# Autodesk Inventor assembly: COMPONENTS
(part 3 of 5)
- C:\Users\Zara\Documents\hera-cad\Node\SNAP V2 enclosure release - pack-n-go export\SNAP V2 enclosure release - pack-n-go export\Workspaces\Workspace\drawings\SNAP Ver2 pack-n-go\Workgroups\NotInProject\CAPAE830X1050D995DD305L335N_C237.ipt
- C:\Users\Zara\Documents\hera-cad\Node\SNAP V2 enclosure release - pack-n-go export\SNAP V2 enclosure release - pack-n-go export\Workspaces\Workspace\drawings\SNAP Ver2 pack-n-go\Workgroups\NotInProject\CAPAE830X1050D995DD305L335N_C244.ipt
- C:\Users\Zara\Documents\hera-cad\Node\SNAP V2 enclosure release - pack-n-go export\SNAP V2 enclosure release - pack-n-go export\Workspaces\Workspace\drawings\SNAP Ver2 pack-n-go\Workgroups\NotInProject\CAPAE830X1050D995DD305L335N_C253.ipt
- C:\Users\Zara\Documents\hera-cad\Node\SNAP V2 enclosure release - pack-n-go export\SNAP V2 enclosure release - pack-n-go export\Workspaces\Workspace\drawings\SNAP Ver2 pack-n-go\Workgroups\NotInProject\CAPAE830X1050D995DD305L335N_C262.ipt
- C:\Users\Zara\Documents\hera-cad\Node\SNAP V2 enclosure release - pack-n-go export\SNAP V2 enclosure release - pack-n-go export\Workspaces\Workspace\drawings\SNAP Ver2 pack-n-go\Workgroups\NotInProject\CAPMP7343X180N-ALT1_C402.ipt
- C:\Users\Zara\Documents\hera-cad\Node\SNAP V2 enclosure release - pack-n-go export\SNAP V2 enclosure release - pack-n-go export\Workspaces\Workspace\drawings\SNAP Ver2 pack-n-go\Workgroups\NotInProject\CAPMP7343X180N-ALT1_C413.ipt
- C:\Users\Zara\Documents\hera-cad\Node\SNAP V2 enclosure release - pack-n-go export\SNAP V2 enclosure release - pack-n-go export\Workspaces\Workspace\drawings\SNAP Ver2 pack-n-go\Workgroups\NotInProject\CAPMP7343X180N-ALT1_C400.ipt
- C:\Users\Zara\Documents\hera-cad\Node\SNAP V2 enclosure release - pack-n-go export\SNAP V2 enclosure release - pack-n-go export\Workspaces\Workspace\drawings\SNAP Ver2 pack-n-go\Workgroups\NotInProject\CAPMP7343X180N-ALT1_C401.ipt
- C:\Users\Zara\Documents\hera-cad\Node\SNAP V2 enclosure release - pack-n-go export\SNAP V2 enclosure release - pack-n-go export\Workspaces\Workspace\drawings\SNAP Ver2 pack-n-go\Workgroups\NotInProject\CAPMP7343X180N-ALT1_C206.ipt
- C:\Users\Zara\Documents\hera-cad\Node\SNAP V2 enclosure release - pack-n-go export\SNAP V2 enclosure release - pack-n-go export\Workspaces\Workspace\drawings\SNAP Ver2 pack-n-go\Workgroups\NotInProject\CAPMP7343X180N-ALT1_C207.ipt
- C:\Users\Zara\Documents\hera-cad\Node\SNAP V2 enclosure release - pack-n-go export\SNAP V2 enclosure release - pack-n-go export\Workspaces\Workspace\drawings\SNAP Ver2 pack-n-go\Workgroups\NotInProject\CAPC2012X140N_C419.ipt
- C:\Users\Zara\Documents\hera-cad\Node\SNAP V2 enclosure release - pack-n-go export\SNAP V2 enclosure release - pack-n-go export\Workspaces\Workspace\drawings\SNAP Ver2 pack-n-go\Workgroups\NotInProject\CAPC2012X140N_C420.ipt
- C:\Users\Zara\Documents\hera-cad\Node\SNAP V2 enclosure release - pack-n-go export\SNAP V2 enclosure release - pack-n-go export\Workspaces\Workspace\drawings\SNAP Ver2 pack-n-go\Workgroups\NotInProject\CAPC2012X140N_C410.ipt
- C:\Users\Zara\Documents\hera-cad\Node\SNAP V2 enclosure release - pack-n-go export\SNAP V2 enclosure release - pack-n-go export\Workspaces\Workspace\drawings\SNAP Ver2 pack-n-go\Workgroups\NotInProject\CAPC2012X140N_C418.ipt
- C:\Users\Zara\Documents\hera-cad\Node\SNAP V2 enclosure release - pack-n-go export\SNAP V2 enclosure release - pack-n-go export\Workspaces\Workspace\drawings\SNAP Ver2 pack-n-go\Workgroups\NotInProject\CAPC2012X140N_C417.ipt
- C:\Users\Zara\Documents\hera-cad\Node\SNAP V2 enclosure release - pack-n-go export\SNAP V2 enclosure release - pack-n-go export\Workspaces\Workspace\drawings\SNAP Ver2 pack-n-go\Workgroups\NotInProject\CAPC2012X140N_C416.ipt
- C:\Users\Zara\Documents\hera-cad\Node\SNAP V2 enclosure release - pack-n-go export\SNAP V2 enclosure release - pack-n-go export\Workspaces\Workspace\drawings\SNAP Ver2 pack-n-go\Workgroups\NotInProject\CAPC2012X140N_C415.ipt
- C:\Users\Zara\Documents\hera-cad\Node\SNAP V2 enclosure release - pack-n-go export\SNAP V2 enclosure release - pack-n-go export\Workspaces\Workspace\drawings\SNAP Ver2 pack-n-go\Workgroups\NotInProject\CAPC2012X140N_C412.ipt
- C:\Users\Zara\Documents\hera-cad\Node\SNAP V2 enclosure release - pack-n-go export\SNAP V2 enclosure release - pack-n-go export\Workspaces\Workspace\drawings\SNAP Ver2 pack-n-go\Workgroups\NotInProject\CAPC2012X140N_C411.ipt
- C:\Users\Zara\Documents\hera-cad\Node\SNAP V2 enclosure release - pack-n-go export\SNAP V2 enclosure release - pack-n-go export\Workspaces\Workspace\drawings\SNAP Ver2 pack-n-go\Workgroups\NotInProject\CAPC2012X140N_C408.ipt
- C:\Users\Zara\Documents\hera-cad\Node\SNAP V2 enclosure release - pack-n-go export\SNAP V2 enclosure release - pack-n-go export\Workspaces\Workspace\drawings\SNAP Ver2 pack-n-go\Workgroups\NotInProject\CAPC2012X140N_C409.ipt
- C:\Users\Zara\Documents\hera-cad\Node\SNAP V2 enclosure release - pack-n-go export\SNAP V2 enclosure release - pack-n-go export\Workspaces\Workspace\drawings\SNAP Ver2 pack-n-go\Workgroups\NotInProject\CAPC2012X140N_C404.ipt
- C:\Users\Zara\Documents\hera-cad\Node\SNAP V2 enclosure release - pack-n-go export\SNAP V2 enclosure release - pack-n-go export\Workspaces\Workspace\drawings\SNAP Ver2 pack-n-go\Workgroups\NotInProject\CAPC2012X140N_C407.ipt
- C:\Users\Zara\Documents\hera-cad\Node\SNAP V2 enclosure release - pack-n-go export\SNAP V2 enclosure release - pack-n-go export\Workspaces\Workspace\drawings\SNAP Ver2 pack-n-go\Workgroups\NotInProject\CAPC2012X140N_C406.ipt
- C:\Users\Zara\Documents\hera-cad\Node\SNAP V2 enclosure release - pack-n-go export\SNAP V2 enclosure release - pack-n-go export\Workspaces\Workspace\drawings\SNAP Ver2 pack-n-go\Workgroups\NotInProject\CAPC2012X140N_C405.ipt
- C:\Users\Zara\Documents\hera-cad\Node\SNAP V2 enclosure release - pack-n-go export\SNAP V2 enclosure release - pack-n-go export\Workspaces\Workspace\drawings\SNAP Ver2 pack-n-go\Workgroups\NotInProject\CAPC2012X140N_C403.ipt
- C:\Users\Zara\Documents\hera-cad\Node\SNAP V2 enclosure release - pack-n-go export\SNAP V2 enclosure release - pack-n-go export\Workspaces\Workspace\drawings\SNAP Ver2 pack-n-go\Workgroups\NotInProject\CAPC2012X140N_C209.ipt
- C:\Users\Zara\Documents\hera-cad\Node\SNAP V2 enclosure release - pack-n-go export\SNAP V2 enclosure release - pack-n-go export\Workspaces\Workspace\drawings\SNAP Ver2 pack-n-go\Workgroups\NotInProject\CAPC2012X140N_C210.ipt
- C:\Users\Zara\Documents\hera-cad\Node\SNAP V2 enclosure release - pack-n-go export\SNAP V2 enclosure release - pack-n-go export\Workspaces\Workspace\drawings\SNAP Ver2 pack-n-go\Workgroups\NotInProject\CAPC2012X140N_C211.ipt
- C:\Users\Zara\Documents\hera-cad\Node\SNAP V2 enclosure release - pack-n-go export\SNAP V2 enclosure release - pack-n-go export\Workspaces\Workspace\drawings\SNAP Ver2 pack-n-go\Workgroups\NotInProject\CAPC2012X140N_C272.ipt
- C:\Users\Zara\Documents\hera-cad\Node\SNAP V2 enclosure release - pack-n-go export\SNAP V2 enclosure release - pack-n-go export\Workspaces\Workspace\drawings\SNAP Ver2 pack-n-go\Workgroups\NotInProject\CAPC2012X140N_C274.ipt
- C:\Users\Zara\Documents\hera-cad\Node\SNAP V2 enclosure release - pack-n-go export\SNAP V2 enclosure release - pack-n-go export\Workspaces\Workspace\drawings\SNAP Ver2 pack-n-go\Workgroups\NotInProject\CAPC2012X140N_C294.ipt
- C:\Users\Zara\Documents\hera-cad\Node\SNAP V2 enclosure release - pack-n-go export\SNAP V2 enclosure release - pack-n-go export\Workspaces\Workspace\drawings\SNAP Ver2 pack-n-go\Workgroups\NotInProject\CAPC2012X140N_C296.ipt
- C:\Users\Zara\Documents\hera-cad\Node\SNAP V2 enclosure release - pack-n-go export\SNAP V2 enclosure release - pack-n-go export\Workspaces\Workspace\drawings\SNAP Ver2 pack-n-go\Workgroups\NotInProject\CAPC2012X140N_C133.ipt
- C:\Users\Zara\Documents\hera-cad\Node\SNAP V2 enclosure release - pack-n-go export\SNAP V2 enclosure release - pack-n-go export\Workspaces\Workspace\drawings\SNAP Ver2 pack-n-go\Workgroups\NotInProject\CAPC2012X140N_C130.ipt
- C:\Users\Zara\Documents\hera-cad\Node\SNAP V2 enclosure release - pack-n-go export\SNAP V2 enclosure release - pack-n-go export\Workspaces\Workspace\drawings\SNAP Ver2 pack-n-go\Workgroups\NotInProject\CAPC2012X140N_C126.ipt
- C:\Users\Zara\Documents\hera-cad\Node\SNAP V2 enclosure release - pack-n-go export\SNAP V2 enclosure release - pack-n-go export\Workspaces\Workspace\drawings\SNAP Ver2 pack-n-go\Workgroups\NotInProject\CAPC2012X140N_C125.ipt
- C:\Users\Zara\Documents\hera-cad\Node\SNAP V2 enclosure release - pack-n-go export\SNAP V2 enclosure release - pack-n-go export\Workspaces\Workspace\drawings\SNAP Ver2 pack-n-go\Workgroups\NotInProject\CAPC2012X140N_C122.ipt
- C:\Users\Zara\Documents\hera-cad\Node\SNAP V2 enclosure release - pack-n-go export\SNAP V2 enclosure release - pack-n-go export\Workspaces\Workspace\drawings\SNAP Ver2 pack-n-go\Workgroups\NotInProject\CAPC2012X140N_C118.ipt
- C:\Users\Zara\Documents\hera-cad\Node\SNAP V2 enclosure release - pack-n-go export\SNAP V2 enclosure release - pack-n-go export\Workspaces\Workspace\drawings\SNAP Ver2 pack-n-go\Workgroups\NotInProject\CAPC0603X30L_C278.ipt
- C:\Users\Zara\Documents\hera-cad\Node\SNAP V2 enclosure release - pack-n-go export\SNAP V2 enclosure release - pack-n-go export\Workspaces\Workspace\drawings\SNAP Ver2 pack-n-go\Workgroups\NotInProject\CAPC0603X30L_C281.ipt
- C:\Users\Zara\Documents\hera-cad\Node\SNAP V2 enclosure release - pack-n-go export\SNAP V2 enclosure release - pack-n-go export\Workspaces\Workspace\drawings\SNAP Ver2 pack-n-go\Workgroups\NotInProject\CAPC0603X30L_C283.ipt
- C:\Users\Zara\Documents\hera-cad\Node\SNAP V2 enclosure release - pack-n-go export\SNAP V2 enclosure release - pack-n-go export\Workspaces\Workspace\drawings\SNAP Ver2 pack-n-go\Workgroups\NotInProject\CAPC0603X30L_C288.ipt
- C:\Users\Zara\Documents\hera-cad\Node\SNAP V2 enclosure release - pack-n-go export\SNAP V2 enclosure release - pack-n-go export\Workspaces\Workspace\drawings\SNAP Ver2 pack-n-go\Workgroups\NotInProject\CAPC0603X30L_C300.ipt
- C:\Users\Zara\Documents\hera-cad\Node\SNAP V2 enclosure release - pack-n-go export\SNAP V2 enclosure release - pack-n-go export\Workspaces\Workspace\drawings\SNAP Ver2 pack-n-go\Workgroups\NotInProject\CAPC0603X30L_C303.ipt
- C:\Users\Zara\Documents\hera-cad\Node\SNAP V2 enclosure release - pack-n-go export\SNAP V2 enclosure release - pack-n-go export\Workspaces\Workspace\drawings\SNAP Ver2 pack-n-go\Workgroups\NotInProject\CAPC0603X30L_C305.ipt
- C:\Users\Zara\Documents\hera-cad\Node\SNAP V2 enclosure release - pack-n-go export\SNAP V2 enclosure release - pack-n-go export\Workspaces\Workspace\drawings\SNAP Ver2 pack-n-go\Workgroups\NotInProject\CAPC0603X30L_C310.ipt
- C:\Users\Zara\Documents\hera-cad\Node\SNAP V2 enclosure release - pack-n-go export\SNAP V2 enclosure release - pack-n-go export\Workspaces\Workspace\drawings\SNAP Ver2 pack-n-go\Workgroups\NotInProject\SOD3717X135_D10.ipt
- C:\Users\Zara\Documents\hera-cad\Node\SNAP V2 enclosure release - pack-n-go export\SNAP V2 enclosure release - pack-n-go export\Workspaces\Workspace\drawings\SNAP Ver2 pack-n-go\Workgroups\NotInProject\SOD3717X135_D9.ipt
- C:\Users\Zara\Documents\hera-cad\Node\SNAP V2 enclosure release - pack-n-go export\SNAP V2 enclosure release - pack-n-go export\Workspaces\Workspace\drawings\SNAP Ver2 pack-n-go\Workgroups\NotInProject\LEDM180X60X60N_DS1.ipt
- C:\Users\Zara\Documents\hera-cad\Node\SNAP V2 enclosure release - pack-n-go export\SNAP V2 enclosure release - pack-n-go export\Workspaces\Workspace\drawings\SNAP Ver2 pack-n-go\Workgroups\NotInProject\LEDM180X60X60N_DS10.ipt
- C:\Users\Zara\Documents\hera-cad\Node\SNAP V2 enclosure release - pack-n-go export\SNAP V2 enclosure release - pack-n-go export\Workspaces\Workspace\drawings\SNAP Ver2 pack-n-go\Workgroups\NotInProject\LEDM180X60X60N_DS11.ipt
- C:\Users\Zara\Documents\hera-cad\Node\SNAP V2 enclosure release - pack-n-go export\SNAP V2 enclosure release - pack-n-go export\Workspaces\Workspace\drawings\SNAP Ver2 pack-n-go\Workgroups\NotInProject\LEDM180X60X60N_DS4.ipt
- C:\Users\Zara\Documents\hera-cad\Node\SNAP V2 enclosure release - pack-n-go export\SNAP V2 enclosure release - pack-n-go export\Workspaces\Workspace\drawings\SNAP Ver2 pack-n-go\Workgroups\NotInProject\LEDM180X60X60N_DS5.ipt
- C:\Users\Zara\Documents\hera-cad\Node\SNAP V2 enclosure release - pack-n-go export\SNAP V2 enclosure release - pack-n-go export\Workspaces\Workspace\drawings\SNAP Ver2 pack-n-go\Workgroups\NotInProject\LEDM180X60X60N_DS7.ipt
- C:\Users\Zara\Documents\hera-cad\Node\SNAP V2 enclosure release - pack-n-go export\SNAP V2 enclosure release - pack-n-go export\Workspaces\Workspace\drawings\SNAP Ver2 pack-n-go\Workgroups\NotInProject\LEDM180X60X60N_DS8.ipt
- C:\Users\Zara\Documents\hera-cad\Node\SNAP V2 enclosure release - pack-n-go export\SNAP V2 enclosure release - pack-n-go export\Workspaces\Workspace\drawings\SNAP Ver2 pack-n-go\Workgroups\NotInProject\LEDM180X60X60N_DS9.ipt
- C:\Users\Zara\Documents\hera-cad\Node\SNAP V2 enclosure release - pack-n-go export\SNAP V2 enclosure release - pack-n-go export\Workspaces\Workspace\drawings\SNAP Ver2 pack-n-go\Workgroups\NotInProject\LEDM180X60X60N_DS2.ipt
- C:\Users\Zara\Documents\hera-cad\Node\SNAP V2 enclosure release - pack-n-go export\SNAP V2 enclosure release - pack-n-go export\Workspaces\Workspace\drawings\SNAP Ver2 pack-n-go\Workgroups\NotInProject\LEDM180X60X60N_DS3.ipt
- C:\Users\Zara\Documents\hera-cad\Node\SNAP V2 enclosure release - pack-n-go export\SNAP V2 enclosure release - pack-n-go export\Workspaces\Workspace\drawings\SNAP Ver2 pack-n-go\Workgroups\NotInProject\INDM4532X340N_L1.ipt
- C:\Users\Zara\Documents\hera-cad\Node\SNAP V2 enclosure release - pack-n-go export\SNAP V2 enclosure release - pack-n-go export\Workspaces\Workspace\drawings\SNAP Ver2 pack-n-go\Workgroups\NotInProject\INDM4532X340N_L10.ipt
- C:\Users\Zara\Documents\hera-cad\Node\SNAP V2 enclosure release - pack-n-go export\SNAP V2 enclosure release - pack-n-go export\Workspaces\Workspace\drawings\SNAP Ver2 pack-n-go\Workgroups\NotInProject\INDM4532X340N_L11.ipt
- C:\Users\Zara\Documents\hera-cad\Node\SNAP V2 enclosure release - pack-n-go export\SNAP V2 enclosure release - pack-n-go export\Workspaces\Workspace\drawings\SNAP Ver2 pack-n-go\Workgroups\NotInProject\INDM4532X340N_L12.ipt
- C:\Users\Zara\Documents\hera-cad\Node\SNAP V2 enclosure release - pack-n-go export\SNAP V2 enclosure release - pack-n-go export\Workspaces\Workspace\drawings\SNAP Ver2 pack-n-go\Workgroups\NotInProject\INDM4532X340N_L2.ipt
- C:\Users\Zara\Documents\hera-cad\Node\SNAP V2 enclosure release - pack-n-go export\SNAP V2 enclosure release - pack-n-go export\Workspaces\Workspace\drawings\SNAP Ver2 pack-n-go\Workgroups\NotInProject\INDM4532X340N_L3.ipt
- C:\Users\Zara\Documents\hera-cad\Node\SNAP V2 enclosure release - pack-n-go export\SNAP V2 enclosure release - pack-n-go export\Workspaces\Workspace\drawings\SNAP Ver2 pack-n-go\Workgroups\NotInProject\INDM4532X340N_L4.ipt
- C:\Users\Zara\Documents\hera-cad\Node\SNAP V2 enclosure release - pack-n-go export\SNAP V2 enclosure release - pack-n-go export\Workspaces\Workspace\drawings\SNAP Ver2 pack-n-go\Workgroups\NotInProject\INDM4532X340N_L5.ipt
- C:\Users\Zara\Documents\hera-cad\Node\SNAP V2 enclosure release - pack-n-go export\SNAP V2 enclosure release - pack-n-go export\Workspaces\Workspace\drawings\SNAP Ver2 pack-n-go\Workgroups\NotInProject\INDM4532X340N_L6.ipt
- C:\Users\Zara\Documents\hera-cad\Node\SNAP V2 enclosure release - pack-n-go export\SNAP V2 enclosure release - pack-n-go export\Workspaces\Workspace\drawings\SNAP Ver2 pack-n-go\Workgroups\NotInProject\INDM4532X340N_L8.ipt
- C:\Users\Zara\Documents\hera-cad\Node\SNAP V2 enclosure release - pack-n-go export\SNAP V2 enclosure release - pack-n-go export\Workspaces\Workspace\drawings\SNAP Ver2 pack-n-go\Workgroups\NotInProject\INDM4532X340N_L7.ipt
- C:\Users\Zara\Documents\hera-cad\Node\SNAP V2 enclosure release - pack-n-go export\SNAP V2 enclosure release - pack-n-go export\Workspaces\Workspace\drawings\SNAP Ver2 pack-n-go\Workgroups\NotInProject\INDM4532X340N_L9.ipt
- C:\Users\Zara\Documents\hera-cad\Node\SNAP V2 enclosure release - pack-n-go export\SNAP V2 enclosure release - pack-n-go export\Workspaces\Workspace\drawings\SNAP Ver2 pack-n-go\Workgroups\NotInProject\INDC2012X110N_L14.ipt
- C:\Users\Zara\Documents\hera-cad\Node\SNAP V2 enclosure release - pack-n-go export\SNAP V2 enclosure release - pack-n-go export\Workspaces\Workspace\drawings\SNAP Ver2 pack-n-go\Workgroups\NotInProject\INDC2012X110N_L13.ipt
- C:\Users\Zara\Documents\hera-cad\Node\SNAP V2 enclosure release - pack-n-go export\SNAP V2 enclosure release - pack-n-go export\Workspaces\Workspace\drawings\SNAP Ver2 pack-n-go\Workgroups\NotInProject\INDM9630X305N_L15.ipt
- C:\Users\Zara\Documents\hera-cad\Node\SNAP V2 enclosure release - pack-n-go export\SNAP V2 enclosure release - pack-n-go export\Workspaces\Workspace\drawings\SNAP Ver2 pack-n-go\Workgroups\NotInProject\INDM9630X305N_L16.ipt
- C:\Users\Zara\Documents\hera-cad\Node\SNAP V2 enclosure release - pack-n-go export\SNAP V2 enclosure release - pack-n-go export\Workspaces\Workspace\drawings\SNAP Ver2 pack-n-go\Workgroups\NotInProject\INDM9630X305N_L17.ipt
- C:\Users\Zara\Documents\hera-cad\Node\SNAP V2 enclosure release - pack-n-go export\SNAP V2 enclosure release - pack-n-go export\Workspaces\Workspace\drawings\SNAP Ver2 pack-n-go\Workgroups\NotInProject\INDM9630X305N_L18.ipt
- C:\Users\Zara\Documents\hera-cad\Node\SNAP V2 enclosure release - pack-n-go export\SNAP V2 enclosure release - pack-n-go export\Workspaces\Workspace\drawings\SNAP Ver2 pack-n-go\Workgroups\NotInProject\INDM9630X305N_L19.ipt
- C:\Users\Zara\Documents\hera-cad\Node\SNAP V2 enclosure release - pack-n-go export\SNAP V2 enclosure release - pack-n-go export\Workspaces\Workspace\drawings\SNAP Ver2 pack-n-go\Workgroups\NotInProject\INDC1608X95L-ALT1_L20.ipt
- C:\Users\Zara\Documents\hera-cad\Node\SNAP V2 enclosure release - pack-n-go export\SNAP V2 enclosure release - pack-n-go export\Workspaces\Workspace\drawings\SNAP Ver2 pack-n-go\Workgroups\NotInProject\INDC1608X95L-ALT1_L21.ipt
- C:\Users\Zara\Documents\hera-cad\Node\SNAP V2 enclosure release - pack-n-go export\SNAP V2 enclosure release - pack-n-go export\Workspaces\Workspace\drawings\SNAP Ver2 pack-n-go\Workgroups\NotInProject\INDC1608X95L-ALT1_L23.ipt
- C:\Users\Zara\Documents\hera-cad\Node\SNAP V2 enclosure release - pack-n-go export\SNAP V2 enclosure release - pack-n-go export\Workspaces\Workspace\drawings\SNAP Ver2 pack-n-go\Workgroups\NotInProject\INDC1608X95L-ALT1_L22.ipt
- C:\Users\Zara\Documents\hera-cad\Node\SNAP V2 enclosure release - pack-n-go export\SNAP V2 enclosure release - pack-n-go export\Workspaces\Workspace\drawings\SNAP Ver2 pack-n-go\Workgroups\NotInProject\INDM5551X200N_L24.ipt
- C:\Users\Zara\Documents\hera-cad\Node\SNAP V2 enclosure release - pack-n-go export\SNAP V2 enclosure release - pack-n-go export\Workspaces\Workspace\drawings\SNAP Ver2 pack-n-go\Workgroups\NotInProject\INDM5551X200N_L25.ipt
- C:\Users\Zara\Documents\hera-cad\Node\SNAP V2 enclosure release - pack-n-go export\SNAP V2 enclosure release - pack-n-go export\Workspaces\Workspace\drawings\SNAP Ver2 pack-n-go\Workgroups\NotInProject\INDM5551X200N_L26.ipt
- C:\Users\Zara\Documents\hera-cad\Node\SNAP V2 enclosure release - pack-n-go export\SNAP V2 enclosure release - pack-n-go export\Workspaces\Workspace\drawings\SNAP Ver2 pack-n-go\Workgroups\NotInProject\INDM5551X200N_L27.ipt
- C:\Users\Zara\Documents\hera-cad\Node\SNAP V2 enclosure release - pack-n-go export\SNAP V2 enclosure release - pack-n-go export\Workspaces\Workspace\drawings\SNAP Ver2 pack-n-go\Workgroups\NotInProject\RESC1005X35N_R443.ipt
- C:\Users\Zara\Documents\hera-cad\Node\SNAP V2 enclosure release - pack-n-go export\SNAP V2 enclosure release - pack-n-go export\Workspaces\Workspace\drawings\SNAP Ver2 pack-n-go\Workgroups\NotInProject\RESC1005X35N_R442.ipt
- C:\Users\Zara\Documents\hera-cad\Node\SNAP V2 enclosure release - pack-n-go export\SNAP V2 enclosure release - pack-n-go export\Workspaces\Workspace\drawings\SNAP Ver2 pack-n-go\Workgroups\NotInProject\RESC1005X35N_R438.ipt
- C:\Users\Zara\Documents\hera-cad\Node\SNAP V2 enclosure release - pack-n-go export\SNAP V2 enclosure release - pack-n-go export\Workspaces\Workspace\drawings\SNAP Ver2 pack-n-go\Workgroups\NotInProject\RESC1005X35N_R437.ipt
- C:\Users\Zara\Documents\hera-cad\Node\SNAP V2 enclosure release - pack-n-go export\SNAP V2 enclosure release - pack-n-go export\Workspaces\Workspace\drawings\SNAP Ver2 pack-n-go\Workgroups\NotInProject\RESC1005X35N_R436.ipt
- C:\Users\Zara\Documents\hera-cad\Node\SNAP V2 enclosure release - pack-n-go export\SNAP V2 enclosure release - pack-n-go export\Workspaces\Workspace\drawings\SNAP Ver2 pack-n-go\Workgroups\NotInProject\RESC1005X35N_R434.ipt
- C:\Users\Zara\Documents\hera-cad\Node\SNAP V2 enclosure release - pack-n-go export\SNAP V2 enclosure release - pack-n-go export\Workspaces\Workspace\drawings\SNAP Ver2 pack-n-go\Workgroups\NotInProject\RESC1005X35N_R114.ipt
- C:\Users\Zara\Documents\hera-cad\Node\SNAP V2 enclosure release - pack-n-go export\SNAP V2 enclosure release - pack-n-go export\Workspaces\Workspace\drawings\SNAP Ver2 pack-n-go\Workgroups\NotInProject\RESC1005X35N_R133.ipt
- C:\Users\Zara\Documents\hera-cad\Node\SNAP V2 enclosure release - pack-n-go export\SNAP V2 enclosure release - pack-n-go export\Workspaces\Workspace\drawings\SNAP Ver2 pack-n-go\Workgroups\NotInProject\RESC1005X35N_R135.ipt
- C:\Users\Zara\Documents\hera-cad\Node\SNAP V2 enclosure release - pack-n-go export\SNAP V2 enclosure release - pack-n-go export\Workspaces\Workspace\drawings\SNAP Ver2 pack-n-go\Workgroups\NotInProject\RESC1005X35N_R139.ipt
- C:\Users\Zara\Documents\hera-cad\Node\SNAP V2 enclosure release - pack-n-go export\SNAP V2 enclosure release - pack-n-go export\Workspaces\Workspace\drawings\SNAP Ver2 pack-n-go\Workgroups\NotInProject\RESC1005X35N_R432.ipt
- C:\Users\Zara\Documents\hera-cad\Node\SNAP V2 enclosure release - pack-n-go export\SNAP V2 enclosure release - pack-n-go export\Workspaces\Workspace\drawings\SNAP Ver2 pack-n-go\Workgroups\NotInProject\RESC1005X35N_R431.ipt
- C:\Users\Zara\Documents\hera-cad\Node\SNAP V2 enclosure release - pack-n-go export\SNAP V2 enclosure release - pack-n-go export\Workspaces\Workspace\drawings\SNAP Ver2 pack-n-go\Workgroups\NotInProject\RESC1005X35N_R427.ipt
- C:\Users\Zara\Documents\hera-cad\Node\SNAP V2 enclosure release - pack-n-go export\SNAP V2 enclosure release - pack-n-go export\Workspaces\Workspace\drawings\SNAP Ver2 pack-n-go\Workgroups\NotInProject\RESC1005X35N_R426.ipt
- C:\Users\Zara\Documents\hera-cad\Node\SNAP V2 enclosure release - pack-n-go export\SNAP V2 enclosure release - pack-n-go export\Workspaces\Workspace\drawings\SNAP Ver2 pack-n-go\Workgroups\NotInProject\RESC1005X35N_R424.ipt
- C:\Users\Zara\Documents\hera-cad\Node\SNAP V2 enclosure release - pack-n-go export\SNAP V2 enclosure release - pack-n-go export\Workspaces\Workspace\drawings\SNAP Ver2 pack-n-go\Workgroups\NotInProject\RESC1005X35N_R423.ipt
- C:\Users\Zara\Documents\hera-cad\Node\SNAP V2 enclosure release - pack-n-go export\SNAP V2 enclosure release - pack-n-go export\Workspaces\Workspace\drawings\SNAP Ver2 pack-n-go\Workgroups\NotInProject\RESC1005X35N_R421.ipt
- C:\Users\Zara\Documents\hera-cad\Node\SNAP V2 enclosure release - pack-n-go export\SNAP V2 enclosure release - pack-n-go export\Workspaces\Workspace\drawings\SNAP Ver2 pack-n-go\Workgroups\NotInProject\RESC1005X35N_R420.ipt
- C:\Users\Zara\Documents\hera-cad\Node\SNAP V2 enclosure release - pack-n-go export\SNAP V2 enclosure release - pack-n-go export\Workspaces\Workspace\drawings\SNAP Ver2 pack-n-go\Workgroups\NotInProject\RESC1005X35N_R433.ipt
- C:\Users\Zara\Documents\hera-cad\Node\SNAP V2 enclosure release - pack-n-go export\SNAP V2 enclosure release - pack-n-go export\Workspaces\Workspace\drawings\SNAP Ver2 pack-n-go\Workgroups\NotInProject\RESC1005X35N_R428.ipt
- C:\Users\Zara\Documents\hera-cad\Node\SNAP V2 enclosure release - pack-n-go export\SNAP V2 enclosure release - pack-n-go export\Workspaces\Workspace\drawings\SNAP Ver2 pack-n-go\Workgroups\NotInProject\RESC1005X35N_R425.ipt
- C:\Users\Zara\Documents\hera-cad\Node\SNAP V2 enclosure release - pack-n-go export\SNAP V2 enclosure release - pack-n-go export\Workspaces\Workspace\drawings\SNAP Ver2 pack-n-go\Workgroups\NotInProject\RESC1005X35N_R422.ipt
- C:\Users\Zara\Documents\hera-cad\Node\SNAP V2 enclosure release - pack-n-go export\SNAP V2 enclosure release - pack-n-go export\Workspaces\Workspace\drawings\SNAP Ver2 pack-n-go\Workgroups\NotInProject\RESC1005X35N_R1.ipt
- C:\Users\Zara\Documents\hera-cad\Node\SNAP V2 enclosure release - pack-n-go export\SNAP V2 enclosure release - pack-n-go export\Workspaces\Workspace\drawings\SNAP Ver2 pack-n-go\Workgroups\NotInProject\RESC1005X35N_R12.ipt
- C:\Users\Zara\Documents\hera-cad\Node\SNAP V2 enclosure release - pack-n-go export\SNAP V2 enclosure release - pack-n-go export\Workspaces\Workspace\drawings\SNAP Ver2 pack-n-go\Workgroups\NotInProject\RESC1005X35N_R13.ipt
- C:\Users\Zara\Documents\hera-cad\Node\SNAP V2 enclosure release - pack-n-go export\SNAP V2 enclosure release - pack-n-go export\Workspaces\Workspace\drawings\SNAP Ver2 pack-n-go\Workgroups\NotInProject\RESC1005X35N_R16.ipt
- C:\Users\Zara\Documents\hera-cad\Node\SNAP V2 enclosure release - pack-n-go export\SNAP V2 enclosure release - pack-n-go export\Workspaces\Workspace\drawings\SNAP Ver2 pack-n-go\Workgroups\NotInProject\RESC1005X35N_R21.ipt
- C:\Users\Zara\Documents\hera-cad\Node\SNAP V2 enclosure release - pack-n-go export\SNAP V2 enclosure release - pack-n-go export\Workspaces\Workspace\drawings\SNAP Ver2 pack-n-go\Workgroups\NotInProject\RESC1005X35N_R25.ipt
- C:\Users\Zara\Documents\hera-cad\Node\SNAP V2 enclosure release - pack-n-go export\SNAP V2 enclosure release - pack-n-go export\Workspaces\Workspace\drawings\SNAP Ver2 pack-n-go\Workgroups\NotInProject\RESC1005X35N_R26.ipt
- C:\Users\Zara\Documents\hera-cad\Node\SNAP V2 enclosure release - pack-n-go export\SNAP V2 enclosure release - pack-n-go export\Workspaces\Workspace\drawings\SNAP Ver2 pack-n-go\Workgroups\NotInProject\RESC1005X35N_R28.ipt
- C:\Users\Zara\Documents\hera-cad\Node\SNAP V2 enclosure release - pack-n-go export\SNAP V2 enclosure release - pack-n-go export\Workspaces\Workspace\drawings\SNAP Ver2 pack-n-go\Workgroups\NotInProject\RESC1005X35N_R29.ipt
- C:\Users\Zara\Documents\hera-cad\Node\SNAP V2 enclosure release - pack-n-go export\SNAP V2 enclosure release - pack-n-go export\Workspaces\Workspace\drawings\SNAP Ver2 pack-n-go\Workgroups\NotInProject\RESC1005X35N_R32.ipt
- C:\Users\Zara\Documents\hera-cad\Node\SNAP V2 enclosure release - pack-n-go export\SNAP V2 enclosure release - pack-n-go export\Workspaces\Workspace\drawings\SNAP Ver2 pack-n-go\Workgroups\NotInProject\RESC1005X35N_R33.ipt
- C:\Users\Zara\Documents\hera-cad\Node\SNAP V2 enclosure release - pack-n-go export\SNAP V2 enclosure release - pack-n-go export\Workspaces\Workspace\drawings\SNAP Ver2 pack-n-go\Workgroups\NotInProject\RESC1005X35N_R36.ipt
- C:\Users\Zara\Documents\hera-cad\Node\SNAP V2 enclosure release - pack-n-go export\SNAP V2 enclosure release - pack-n-go export\Workspaces\Workspace\drawings\SNAP Ver2 pack-n-go\Workgroups\NotInProject\RESC1005X35N_R41.ipt
- C:\Users\Zara\Documents\hera-cad\Node\SNAP V2 enclosure release - pack-n-go export\SNAP V2 enclosure release - pack-n-go export\Workspaces\Workspace\drawings\SNAP Ver2 pack-n-go\Workgroups\NotInProject\RESC1005X35N_R45.ipt
- C:\Users\Zara\Documents\hera-cad\Node\SNAP V2 enclosure release - pack-n-go export\SNAP V2 enclosure release - pack-n-go export\Workspaces\Workspace\drawings\SNAP Ver2 pack-n-go\Workgroups\NotInProject\RESC1005X35N_R46.ipt
- C:\Users\Zara\Documents\hera-cad\Node\SNAP V2 enclosure release - pack-n-go export\SNAP V2 enclosure release - pack-n-go export\Workspaces\Workspace\drawings\SNAP Ver2 pack-n-go\Workgroups\NotInProject\RESC1005X35N_R48.ipt
- C:\Users\Zara\Documents\hera-cad\Node\SNAP V2 enclosure release - pack-n-go export\SNAP V2 enclosure release - pack-n-go export\Workspaces\Workspace\drawings\SNAP Ver2 pack-n-go\Workgroups\NotInProject\RESC1005X35N_R49.ipt
- C:\Users\Zara\Documents\hera-cad\Node\SNAP V2 enclosure release - pack-n-go export\SNAP V2 enclosure release - pack-n-go export\Workspaces\Workspace\drawings\SNAP Ver2 pack-n-go\Workgroups\NotInProject\RESC1005X35N_R5.ipt
- C:\Users\Zara\Documents\hera-cad\Node\SNAP V2 enclosure release - pack-n-go export\SNAP V2 enclosure release - pack-n-go export\Workspaces\Workspace\drawings\SNAP Ver2 pack-n-go\Workgroups\NotInProject\RESC1005X35N_R52.ipt
- C:\Users\Zara\Documents\hera-cad\Node\SNAP V2 enclosure release - pack-n-go export\SNAP V2 enclosure release - pack-n-go export\Workspaces\Workspace\drawings\SNAP Ver2 pack-n-go\Workgroups\NotInProject\RESC1005X35N_R53.ipt
- C:\Users\Zara\Documents\hera-cad\Node\SNAP V2 enclosure release - pack-n-go export\SNAP V2 enclosure release - pack-n-go export\Workspaces\Workspace\drawings\SNAP Ver2 pack-n-go\Workgroups\NotInProject\RESC1005X35N_R56.ipt
- C:\Users\Zara\Documents\hera-cad\Node\SNAP V2 enclosure release - pack-n-go export\SNAP V2 enclosure release - pack-n-go export\Workspaces\Workspace\drawings\SNAP Ver2 pack-n-go\Workgroups\NotInProject\RESC1005X35N_R6.ipt
- C:\Users\Zara\Documents\hera-cad\Node\SNAP V2 enclosure release - pack-n-go export\SNAP V2 enclosure release - pack-n-go export\Workspaces\Workspace\drawings\SNAP Ver2 pack-n-go\Workgroups\NotInProject\RESC1005X35N_R8.ipt
- C:\Users\Zara\Documents\hera-cad\Node\SNAP V2 enclosure release - pack-n-go export\SNAP V2 enclosure release - pack-n-go export\Workspaces\Workspace\drawings\SNAP Ver2 pack-n-go\Workgroups\NotInProject\RESC1005X35N_R9.ipt
- C:\Users\Zara\Documents\hera-cad\Node\SNAP V2 enclosure release - pack-n-go export\SNAP V2 enclosure release - pack-n-go export\Workspaces\Workspace\drawings\SNAP Ver2 pack-n-go\Workgroups\NotInProject\RESC1005X35N_R10.ipt
- C:\Users\Zara\Documents\hera-cad\Node\SNAP V2 enclosure release - pack-n-go export\SNAP V2 enclosure release - pack-n-go export\Workspaces\Workspace\drawings\SNAP Ver2 pack-n-go\Workgroups\NotInProject\RESC1005X35N_R14.ipt
- C:\Users\Zara\Documents\hera-cad\Node\SNAP V2 enclosure release - pack-n-go export\SNAP V2 enclosure release - pack-n-go export\Workspaces\Workspace\drawings\SNAP Ver2 pack-n-go\Workgroups\NotInProject\RESC1005X35N_R2.ipt
- C:\Users\Zara\Documents\hera-cad\Node\SNAP V2 enclosure release - pack-n-go export\SNAP V2 enclosure release - pack-n-go export\Workspaces\Workspace\drawings\SNAP Ver2 pack-n-go\Workgroups\NotInProject\RESC1005X35N_R22.ipt
- C:\Users\Zara\Documents\hera-cad\Node\SNAP V2 enclosure release - pack-n-go export\SNAP V2 enclosure release - pack-n-go export\Workspaces\Workspace\drawings\SNAP Ver2 pack-n-go\Workgroups\NotInProject\RESC1005X35N_R24.ipt
- C:\Users\Zara\Documents\hera-cad\Node\SNAP V2 enclosure release - pack-n-go export\SNAP V2 enclosure release - pack-n-go export\Workspaces\Workspace\drawings\SNAP Ver2 pack-n-go\Workgroups\NotInProject\RESC1005X35N_R30.ipt
- C:\Users\Zara\Documents\hera-cad\Node\SNAP V2 enclosure release - pack-n-go export\SNAP V2 enclosure release - pack-n-go export\Workspaces\Workspace\drawings\SNAP Ver2 pack-n-go\Workgroups\NotInProject\RESC1005X35N_R34.ipt
- C:\Users\Zara\Documents\hera-cad\Node\SNAP V2 enclosure release - pack-n-go export\SNAP V2 enclosure release - pack-n-go export\Workspaces\Workspace\drawings\SNAP Ver2 pack-n-go\Workgroups\NotInProject\RESC1005X35N_R4.ipt
- C:\Users\Zara\Documents\hera-cad\Node\SNAP V2 enclosure release - pack-n-go export\SNAP V2 enclosure release - pack-n-go export\Workspaces\Workspace\drawings\SNAP Ver2 pack-n-go\Workgroups\NotInProject\RESC1005X35N_R42.ipt
- C:\Users\Zara\Documents\hera-cad\Node\SNAP V2 enclosure release - pack-n-go export\SNAP V2 enclosure release - pack-n-go export\Workspaces\Workspace\drawings\SNAP Ver2 pack-n-go\Workgroups\NotInProject\RESC1005X35N_R44.ipt
- C:\Users\Zara\Documents\hera-cad\Node\SNAP V2 enclosure release - pack-n-go export\SNAP V2 enclosure release - pack-n-go export\Workspaces\Workspace\drawings\SNAP Ver2 pack-n-go\Workgroups\NotInProject\RESC1005X35N_R50.ipt
- C:\Users\Zara\Documents\hera-cad\Node\SNAP V2 enclosure release - pack-n-go export\SNAP V2 enclosure release - pack-n-go export\Workspaces\Workspace\drawings\SNAP Ver2 pack-n-go\Workgroups\NotInProject\RESC1005X35N_R54.ipt
- C:\Users\Zara\Documents\hera-cad\Node\SNAP V2 enclosure release - pack-n-go export\SNAP V2 enclosure release - pack-n-go export\Workspaces\Workspace\drawings\SNAP Ver2 pack-n-go\Workgroups\NotInProject\RESC1005X35N_R100.ipt
- C:\Users\Zara\Documents\hera-cad\Node\SNAP V2 enclosure release - pack-n-go export\SNAP V2 enclosure release - pack-n-go export\Workspaces\Workspace\drawings\SNAP Ver2 pack-n-go\Workgroups\NotInProject\RESC1005X35N_R102.ipt
- C:\Users\Zara\Documents\hera-cad\Node\SNAP V2 enclosure release - pack-n-go export\SNAP V2 enclosure release - pack-n-go export\Workspaces\Workspace\drawings\SNAP Ver2 pack-n-go\Workgroups\NotInProject\RESC1005X35N_R103.ipt
- C:\Users\Zara\Documents\hera-cad\Node\SNAP V2 enclosure release - pack-n-go export\SNAP V2 enclosure release - pack-n-go export\Workspaces\Workspace\drawings\SNAP Ver2 pack-n-go\Workgroups\NotInProject\RESC1005X35N_R104.ipt
- C:\Users\Zara\Documents\hera-cad\Node\SNAP V2 enclosure release - pack-n-go export\SNAP V2 enclosure release - pack-n-go export\Workspaces\Workspace\drawings\SNAP Ver2 pack-n-go\Workgroups\NotInProject\RESC1005X35N_R105.ipt
- C:\Users\Zara\Documents\hera-cad\Node\SNAP V2 enclosure release - pack-n-go export\SNAP V2 enclosure release - pack-n-go export\Workspaces\Workspace\drawings\SNAP Ver2 pack-n-go\Workgroups\NotInProject\RESC1005X35N_R106.ipt
- C:\Users\Zara\Documents\hera-cad\Node\SNAP V2 enclosure release - pack-n-go export\SNAP V2 enclosure release - pack-n-go export\Workspaces\Workspace\drawings\SNAP Ver2 pack-n-go\Workgroups\NotInProject\RESC1005X35N_R96.ipt
- C:\Users\Zara\Documents\hera-cad\Node\SNAP V2 enclosure release - pack-n-go export\SNAP V2 enclosure release - pack-n-go export\Workspaces\Workspace\drawings\SNAP Ver2 pack-n-go\Workgroups\NotInProject\RESC1005X35N_R97.ipt
- C:\Users\Zara\Documents\hera-cad\Node\SNAP V2 enclosure release - pack-n-go export\SNAP V2 enclosure release - pack-n-go export\Workspaces\Workspace\drawings\SNAP Ver2 pack-n-go\Workgroups\NotInProject\RESC1005X35N_R109.ipt
- C:\Users\Zara\Documents\hera-cad\Node\SNAP V2 enclosure release - pack-n-go export\SNAP V2 enclosure release - pack-n-go export\Workspaces\Workspace\drawings\SNAP Ver2 pack-n-go\Workgroups\NotInProject\RESC1005X35N_R140.ipt
- C:\Users\Zara\Documents\hera-cad\Node\SNAP V2 enclosure release - pack-n-go export\SNAP V2 enclosure release - pack-n-go export\Workspaces\Workspace\drawings\SNAP Ver2 pack-n-go\Workgroups\NotInProject\RESC1005X35N_R145.ipt
- C:\Users\Zara\Documents\hera-cad\Node\SNAP V2 enclosure release - pack-n-go export\SNAP V2 enclosure release - pack-n-go export\Workspaces\Workspace\drawings\SNAP Ver2 pack-n-go\Workgroups\NotInProject\RESC1005X35N_R146.ipt
- C:\Users\Zara\Documents\hera-cad\Node\SNAP V2 enclosure release - pack-n-go export\SNAP V2 enclosure release - pack-n-go export\Workspaces\Workspace\drawings\SNAP Ver2 pack-n-go\Workgroups\NotInProject\RESC1005X35N_R147.ipt
- C:\Users\Zara\Documents\hera-cad\Node\SNAP V2 enclosure release - pack-n-go export\SNAP V2 enclosure release - pack-n-go export\Workspaces\Workspace\drawings\SNAP Ver2 pack-n-go\Workgroups\NotInProject\RESC1005X35N_R148.ipt
- C:\Users\Zara\Documents\hera-cad\Node\SNAP V2 enclosure release - pack-n-go export\SNAP V2 enclosure release - pack-n-go export\Workspaces\Workspace\drawings\SNAP Ver2 pack-n-go\Workgroups\NotInProject\RESC1005X35N_R154.ipt
- C:\Users\Zara\Documents\hera-cad\Node\SNAP V2 enclosure release - pack-n-go export\SNAP V2 enclosure release - pack-n-go export\Workspaces\Workspace\drawings\SNAP Ver2 pack-n-go\Workgroups\NotInProject\RESC1005X35N_R157.ipt
- C:\Users\Zara\Documents\hera-cad\Node\SNAP V2 enclosure release - pack-n-go export\SNAP V2 enclosure release - pack-n-go export\Workspaces\Workspace\drawings\SNAP Ver2 pack-n-go\Workgroups\NotInProject\RESC1005X35N_R158.ipt
- C:\Users\Zara\Documents\hera-cad\Node\SNAP V2 enclosure release - pack-n-go export\SNAP V2 enclosure release - pack-n-go export\Workspaces\Workspace\drawings\SNAP Ver2 pack-n-go\Workgroups\NotInProject\RESC1005X35N_R159.ipt
- C:\Users\Zara\Documents\hera-cad\Node\SNAP V2 enclosure release - pack-n-go export\SNAP V2 enclosure release - pack-n-go export\Workspaces\Workspace\drawings\SNAP Ver2 pack-n-go\Workgroups\NotInProject\RESC1005X35N_R160.ipt
- C:\Users\Zara\Documents\hera-cad\Node\SNAP V2 enclosure release - pack-n-go export\SNAP V2 enclosure release - pack-n-go export\Workspaces\Workspace\drawings\SNAP Ver2 pack-n-go\Workgroups\NotInProject\RESC1005X35N_R161.ipt
- C:\Users\Zara\Documents\hera-cad\Node\SNAP V2 enclosure release - pack-n-go export\SNAP V2 enclosure release - pack-n-go export\Workspaces\Workspace\drawings\SNAP Ver2 pack-n-go\Workgroups\NotInProject\RESC1005X35N_R162.ipt
- C:\Users\Zara\Documents\hera-cad\Node\SNAP V2 enclosure release - pack-n-go export\SNAP V2 enclosure release - pack-n-go export\Workspaces\Workspace\drawings\SNAP Ver2 pack-n-go\Workgroups\NotInProject\RESC1005X35N_R163.ipt
- C:\Users\Zara\Documents\hera-cad\Node\SNAP V2 enclosure release - pack-n-go export\SNAP V2 enclosure release - pack-n-go export\Workspaces\Workspace\drawings\SNAP Ver2 pack-n-go\Workgroups\NotInProject\RESC1005X35N_R164.ipt
- C:\Users\Zara\Documents\hera-cad\Node\SNAP V2 enclosure release - pack-n-go export\SNAP V2 enclosure release - pack-n-go export\Workspaces\Workspace\drawings\SNAP Ver2 pack-n-go\Workgroups\NotInProject\RESC1005X35N_R194.ipt
- C:\Users\Zara\Documents\hera-cad\Node\SNAP V2 enclosure release - pack-n-go export\SNAP V2 enclosure release - pack-n-go export\Workspaces\Workspace\drawings\SNAP Ver2 pack-n-go\Workgroups\NotInProject\RESC1005X35N_R195.ipt
- C:\Users\Zara\Documents\hera-cad\Node\SNAP V2 enclosure release - pack-n-go export\SNAP V2 enclosure release - pack-n-go export\Workspaces\Workspace\drawings\SNAP Ver2 pack-n-go\Workgroups\NotInProject\RESC1005X35N_R196.ipt
- C:\Users\Zara\Documents\hera-cad\Node\SNAP V2 enclosure release - pack-n-go export\SNAP V2 enclosure release - pack-n-go export\Workspaces\Workspace\drawings\SNAP Ver2 pack-n-go\Workgroups\NotInProject\RESC1005X35N_R201.ipt
- C:\Users\Zara\Documents\hera-cad\Node\SNAP V2 enclosure release - pack-n-go export\SNAP V2 enclosure release - pack-n-go export\Workspaces\Workspace\drawings\SNAP Ver2 pack-n-go\Workgroups\NotInProject\RESC1005X35N_R202.ipt
- C:\Users\Zara\Documents\hera-cad\Node\SNAP V2 enclosure release - pack-n-go export\SNAP V2 enclosure release - pack-n-go export\Workspaces\Workspace\drawings\SNAP Ver2 pack-n-go\Workgroups\NotInProject\RESC1005X35N_R203.ipt
- C:\Users\Zara\Documents\hera-cad\Node\SNAP V2 enclosure release - pack-n-go export\SNAP V2 enclosure release - pack-n-go export\Workspaces\Workspace\drawings\SNAP Ver2 pack-n-go\Workgroups\NotInProject\RESC1005X35N_R204.ipt
- C:\Users\Zara\Documents\hera-cad\Node\SNAP V2 enclosure release - pack-n-go export\SNAP V2 enclosure release - pack-n-go export\Workspaces\Workspace\drawings\SNAP Ver2 pack-n-go\Workgroups\NotInProject\RESC1005X35N_R205.ipt
- C:\Users\Zara\Documents\hera-cad\Node\SNAP V2 enclosure release - pack-n-go export\SNAP V2 enclosure release - pack-n-go export\Workspaces\Workspace\drawings\SNAP Ver2 pack-n-go\Workgroups\NotInProject\RESC1005X35N_R206.ipt
- C:\Users\Zara\Documents\hera-cad\Node\SNAP V2 enclosure release - pack-n-go export\SNAP V2 enclosure release - pack-n-go export\Workspaces\Workspace\drawings\SNAP Ver2 pack-n-go\Workgroups\NotInProject\RESC1005X35N_R207.ipt
- C:\Users\Zara\Documents\hera-cad\Node\SNAP V2 enclosure release - pack-n-go export\SNAP V2 enclosure release - pack-n-go export\Workspaces\Workspace\drawings\SNAP Ver2 pack-n-go\Workgroups\NotInProject\RESC1005X35N_R208.ipt
- C:\Users\Zara\Documents\hera-cad\Node\SNAP V2 enclosure release - pack-n-go export\SNAP V2 enclosure release - pack-n-go export\Workspaces\Workspace\drawings\SNAP Ver2 pack-n-go\Workgroups\NotInProject\RESC1005X35N_R210.ipt
- C:\Users\Zara\Documents\hera-cad\Node\SNAP V2 enclosure release - pack-n-go export\SNAP V2 enclosure release - pack-n-go export\Workspaces\Workspace\drawings\SNAP Ver2 pack-n-go\Workgroups\NotInProject\RESC1005X35N_R211.ipt
- C:\Users\Zara\Documents\hera-cad\Node\SNAP V2 enclosure release - pack-n-go export\SNAP V2 enclosure release - pack-n-go export\Workspaces\Workspace\drawings\SNAP Ver2 pack-n-go\Workgroups\NotInProject\RESC1005X35N_R212.ipt
- C:\Users\Zara\Documents\hera-cad\Node\SNAP V2 enclosure release - pack-n-go export\SNAP V2 enclosure release - pack-n-go export\Workspaces\Workspace\drawings\SNAP Ver2 pack-n-go\Workgroups\NotInProject\RESC1005X35N_R213.ipt
- C:\Users\Zara\Documents\hera-cad\Node\SNAP V2 enclosure release - pack-n-go export\SNAP V2 enclosure release - pack-n-go export\Workspaces\Workspace\drawings\SNAP Ver2 pack-n-go\Workgroups\NotInProject\RESC1005X35N_R214.ipt
- C:\Users\Zara\Documents\hera-cad\Node\SNAP V2 enclosure release - pack-n-go export\SNAP V2 enclosure release - pack-n-go export\Workspaces\Workspace\drawings\SNAP Ver2 pack-n-go\Workgroups\NotInProject\RESC1005X35N_R215.ipt
- C:\Users\Zara\Documents\hera-cad\Node\SNAP V2 enclosure release - pack-n-go export\SNAP V2 enclosure release - pack-n-go export\Workspaces\Workspace\drawings\SNAP Ver2 pack-n-go\Workgroups\NotInProject\RESC1005X35N_R216.ipt
- C:\Users\Zara\Documents\hera-cad\Node\SNAP V2 enclosure release - pack-n-go export\SNAP V2 enclosure release - pack-n-go export\Workspaces\Workspace\drawings\SNAP Ver2 pack-n-go\Workgroups\NotInProject\RESC1005X35N_R217.ipt
- C:\Users\Zara\Documents\hera-cad\Node\SNAP V2 enclosure release - pack-n-go export\SNAP V2 enclosure release - pack-n-go export\Workspaces\Workspace\drawings\SNAP Ver2 pack-n-go\Workgroups\NotInProject\RESC1005X35N_R218.ipt
- C:\Users\Zara\Documents\hera-cad\Node\SNAP V2 enclosure release - pack-n-go export\SNAP V2 enclosure release - pack-n-go export\Workspaces\Workspace\drawings\SNAP Ver2 pack-n-go\Workgroups\NotInProject\RESC1005X35N_R219.ipt
- C:\Users\Zara\Documents\hera-cad\Node\SNAP V2 enclosure release - pack-n-go export\SNAP V2 enclosure release - pack-n-go export\Workspaces\Workspace\drawings\SNAP Ver2 pack-n-go\Workgroups\NotInProject\RESC1005X35N_R221.ipt
- C:\Users\Zara\Documents\hera-cad\Node\SNAP V2 enclosure release - pack-n-go export\SNAP V2 enclosure release - pack-n-go export\Workspaces\Workspace\drawings\SNAP Ver2 pack-n-go\Workgroups\NotInProject\RESC1005X35N_R222.ipt
- C:\Users\Zara\Documents\hera-cad\Node\SNAP V2 enclosure release - pack-n-go export\SNAP V2 enclosure release - pack-n-go export\Workspaces\Workspace\drawings\SNAP Ver2 pack-n-go\Workgroups\NotInProject\RESC1005X35N_R223.ipt
- C:\Users\Zara\Documents\hera-cad\Node\SNAP V2 enclosure release - pack-n-go export\SNAP V2 enclosure release - pack-n-go export\Workspaces\Workspace\drawings\SNAP Ver2 pack-n-go\Workgroups\NotInProject\RESC1005X35N_R224.ipt
- C:\Users\Zara\Documents\hera-cad\Node\SNAP V2 enclosure release - pack-n-go export\SNAP V2 enclosure release - pack-n-go export\Workspaces\Workspace\drawings\SNAP Ver2 pack-n-go\Workgroups\NotInProject\RESC1005X35N_R226.ipt
- C:\Users\Zara\Documents\hera-cad\Node\SNAP V2 enclosure release - pack-n-go export\SNAP V2 enclosure release - pack-n-go export\Workspaces\Workspace\drawings\SNAP Ver2 pack-n-go\Workgroups\NotInProject\RESC1005X35N_R227.ipt
- C:\Users\Zara\Documents\hera-cad\Node\SNAP V2 enclosure release - pack-n-go export\SNAP V2 enclosure release - pack-n-go export\Workspaces\Workspace\drawings\SNAP Ver2 pack-n-go\Workgroups\NotInProject\RESC1005X35N_R11.ipt
- C:\Users\Zara\Documents\hera-cad\Node\SNAP V2 enclosure release - pack-n-go export\SNAP V2 enclosure release - pack-n-go export\Workspaces\Workspace\drawings\SNAP Ver2 pack-n-go\Workgroups\NotInProject\RESC1005X35N_R15.ipt
- C:\Users\Zara\Documents\hera-cad\Node\SNAP V2 enclosure release - pack-n-go export\SNAP V2 enclosure release - pack-n-go export\Workspaces\Workspace\drawings\SNAP Ver2 pack-n-go\Workgroups\NotInProject\RESC1005X35N_R23.ipt
- C:\Users\Zara\Documents\hera-cad\Node\SNAP V2 enclosure release - pack-n-go export\SNAP V2 enclosure release - pack-n-go export\Workspaces\Workspace\drawings\SNAP Ver2 pack-n-go\Workgroups\NotInProject\RESC1005X35N_R27.ipt
- C:\Users\Zara\Documents\hera-cad\Node\SNAP V2 enclosure release - pack-n-go export\SNAP V2 enclosure release - pack-n-go export\Workspaces\Workspace\drawings\SNAP Ver2 pack-n-go\Workgroups\NotInProject\RESC1005X35N_R3.ipt
- C:\Users\Zara\Documents\hera-cad\Node\SNAP V2 enclosure release - pack-n-go export\SNAP V2 enclosure release - pack-n-go export\Workspaces\Workspace\drawings\SNAP Ver2 pack-n-go\Workgroups\NotInProject\RESC1005X35N_R31.ipt
- C:\Users\Zara\Documents\hera-cad\Node\SNAP V2 enclosure release - pack-n-go export\SNAP V2 enclosure release - pack-n-go export\Workspaces\Workspace\drawings\SNAP Ver2 pack-n-go\Workgroups\NotInProject\RESC1005X35N_R35.ipt
- C:\Users\Zara\Documents\hera-cad\Node\SNAP V2 enclosure release - pack-n-go export\SNAP V2 enclosure release - pack-n-go export\Workspaces\Workspace\drawings\SNAP Ver2 pack-n-go\Workgroups\NotInProject\RESC1005X35N_R43.ipt
- C:\Users\Zara\Documents\hera-cad\Node\SNAP V2 enclosure release - pack-n-go export\SNAP V2 enclosure release - pack-n-go export\Workspaces\Workspace\drawings\SNAP Ver2 pack-n-go\Workgroups\NotInProject\RESC1005X35N_R47.ipt
- C:\Users\Zara\Documents\hera-cad\Node\SNAP V2 enclosure release - pack-n-go export\SNAP V2 enclosure release - pack-n-go export\Workspaces\Workspace\drawings\SNAP Ver2 pack-n-go\Workgroups\NotInProject\RESC1005X35N_R51.ipt
- C:\Users\Zara\Documents\hera-cad\Node\SNAP V2 enclosure release - pack-n-go export\SNAP V2 enclosure release - pack-n-go export\Workspaces\Workspace\drawings\SNAP Ver2 pack-n-go\Workgroups\NotInProject\RESC1005X35N_R55.ipt
- C:\Users\Zara\Documents\hera-cad\Node\SNAP V2 enclosure release - pack-n-go export\SNAP V2 enclosure release - pack-n-go export\Workspaces\Workspace\drawings\SNAP Ver2 pack-n-go\Workgroups\NotInProject\RESC1005X35N_R7.ipt
- C:\Users\Zara\Documents\hera-cad\Node\SNAP V2 enclosure release - pack-n-go export\SNAP V2 enclosure release - pack-n-go export\Workspaces\Workspace\drawings\SNAP Ver2 pack-n-go\Workgroups\NotInProject\RESC1005X35N_R110.ipt
- C:\Users\Zara\Documents\hera-cad\Node\SNAP V2 enclosure release - pack-n-go export\SNAP V2 enclosure release - pack-n-go export\Workspaces\Workspace\drawings\SNAP Ver2 pack-n-go\Workgroups\NotInProject\RESC1005X35N_R112.ipt
- C:\Users\Zara\Documents\hera-cad\Node\SNAP V2 enclosure release - pack-n-go export\SNAP V2 enclosure release - pack-n-go export\Workspaces\Workspace\drawings\SNAP Ver2 pack-n-go\Workgroups\NotInProject\RESC1005X35N_R113.ipt
- C:\Users\Zara\Documents\hera-cad\Node\SNAP V2 enclosure release - pack-n-go export\SNAP V2 enclosure release - pack-n-go export\Workspaces\Workspace\drawings\SNAP Ver2 pack-n-go\Workgroups\NotInProject\RESC1005X35N_R115.ipt
- C:\Users\Zara\Documents\hera-cad\Node\SNAP V2 enclosure release - pack-n-go export\SNAP V2 enclosure release - pack-n-go export\Workspaces\Workspace\drawings\SNAP Ver2 pack-n-go\Workgroups\NotInProject\RESC1005X35N_R116.ipt
- C:\Users\Zara\Documents\hera-cad\Node\SNAP V2 enclosure release - pack-n-go export\SNAP V2 enclosure release - pack-n-go export\Workspaces\Workspace\drawings\SNAP Ver2 pack-n-go\Workgroups\NotInProject\RESC1005X35N_R120.ipt
- C:\Users\Zara\Documents\hera-cad\Node\SNAP V2 enclosure release - pack-n-go export\SNAP V2 enclosure release - pack-n-go export\Workspaces\Workspace\drawings\SNAP Ver2 pack-n-go\Workgroups\NotInProject\RESC1005X35N_R124.ipt
- C:\Users\Zara\Documents\hera-cad\Node\SNAP V2 enclosure release - pack-n-go export\SNAP V2 enclosure release - pack-n-go export\Workspaces\Workspace\drawings\SNAP Ver2 pack-n-go\Workgroups\NotInProject\RESC1005X35N_R111.ipt
- C:\Users\Zara\Documents\hera-cad\Node\SNAP V2 enclosure release - pack-n-go export\SNAP V2 enclosure release - pack-n-go export\Workspaces\Workspace\drawings\SNAP Ver2 pack-n-go\Workgroups\NotInProject\RESC1005X35N_R117.ipt
- C:\Users\Zara\Documents\hera-cad\Node\SNAP V2 enclosure release - pack-n-go export\SNAP V2 enclosure release - pack-n-go export\Workspaces\Workspace\drawings\SNAP Ver2 pack-n-go\Workgroups\NotInProject\RESC1005X35N_R119.ipt
- C:\Users\Zara\Documents\hera-cad\Node\SNAP V2 enclosure release - pack-n-go export\SNAP V2 enclosure release - pack-n-go export\Workspaces\Workspace\drawings\SNAP Ver2 pack-n-go\Workgroups\NotInProject\RESC1005X35N_R123.ipt
- C:\Users\Zara\Documents\hera-cad\Node\SNAP V2 enclosure release - pack-n-go export\SNAP V2 enclosure release - pack-n-go export\Workspaces\Workspace\drawings\SNAP Ver2 pack-n-go\Workgroups\NotInProject\RESC1005X35N_R130.ipt
- C:\Users\Zara\Documents\hera-cad\Node\SNAP V2 enclosure release - pack-n-go export\SNAP V2 enclosure release - pack-n-go export\Workspaces\Workspace\drawings\SNAP Ver2 pack-n-go\Workgroups\NotInProject\RESC1005X35N_R132.ipt